# Autodesk Inventor assembly: Sessao7_02_04_2025_999_0001
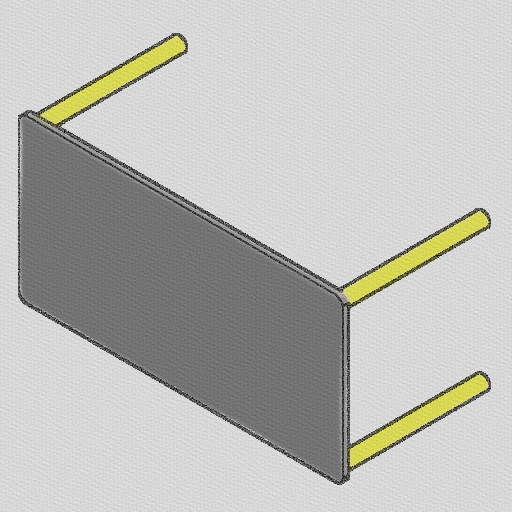
[picture p0: Inventor's stored thumbnail of the model, 512x512]
Saved by Autodesk Inventor 2025.2 (Build 292293000, 293)
## iProperties
Created: 2025-04-02
Part Number: Sessao7_02_04_2025_999_0001
Document SubType Name: Assembly
Designer: lucas
Author: lucas
## Documents named in this file (3)
- C:\Users\lucas\OneDrive\Documentos\Documentos\Gustavo\Mozangao\Robotica_Fundamentos\Inventor\Sessao7_02_04_2025\Sessao7_02_04_2025_999_0001.iam
- C:\Users\lucas\OneDrive\Documentos\Documentos\Gustavo\Mozangao\Robotica_Fundamentos\Inventor\Sessao7_02_04_2025\Sessao7_02_04_2025_0001_001.ipt
- C:\Users\lucas\OneDrive\Documentos\Documentos\Gustavo\Mozangao\Robotica_Fundamentos\Inventor\Sessao7_02_04_2025\Sessao7_02_04_2025_0002_001.ipt
## Components (5 placed, 2 different names)
1. Sessao7_02_04_2025_0001_001:1 — Alinhado:1, Alinhado:2, Alinhado:3, Coincidente:1, Coincidente:2, Coincidente:3, Coincidente:4, Coincidente:5, Alinhado:10, Coincidente:6, Coincidente:7, Coincidente:8, Coincidente:9
2. Sessao7_02_04_2025_0002_001:1 — Coincidente:1, Alinhado:6, Alinhado:7, Alinhado:8, Simetria:1, Simetria:3, Coincidente:5, Alinhado:10, Coincidente:9
3. Sessao7_02_04_2025_0002_001:2 — Coincidente:3, Alinhado:9, Simetria:2, Coincidente:7
4. Sessao7_02_04_2025_0002_001:3 — Coincidente:4, Alinhado:6, Alinhado:7, Simetria:1, Alinhado:9, Simetria:2, Coincidente:8
5. Sessao7_02_04_2025_0002_001:4 — Coincidente:2, Alinhado:8, Simetria:3, Coincidente:6
## Relationships (20: Mate 9, Flush 8, Symmetry 3)
- Alinhado:1 [Flush]: Sessao7_02_04_2025_0001_001:1
- Alinhado:2 [Flush]: Sessao7_02_04_2025_0001_001:1
- Alinhado:3 [Flush]: Sessao7_02_04_2025_0001_001:1
- Coincidente:1 [Mate]: Sessao7_02_04_2025_0001_001:1 ↔ Sessao7_02_04_2025_0002_001:1
- Coincidente:2 [Mate]: Sessao7_02_04_2025_0001_001:1 ↔ Sessao7_02_04_2025_0002_001:4
- Coincidente:3 [Mate]: Sessao7_02_04_2025_0001_001:1 ↔ Sessao7_02_04_2025_0002_001:2
- Coincidente:4 [Mate]: Sessao7_02_04_2025_0001_001:1 ↔ Sessao7_02_04_2025_0002_001:3
- Alinhado:6 [Flush]: Sessao7_02_04_2025_0002_001:1 ↔ Sessao7_02_04_2025_0002_001:3
- Alinhado:7 [Flush]: Sessao7_02_04_2025_0002_001:1 ↔ Sessao7_02_04_2025_0002_001:3
- Alinhado:8 [Flush]: Sessao7_02_04_2025_0002_001:1 ↔ Sessao7_02_04_2025_0002_001:4
- Simetria:1 [Symmetry]: Sessao7_02_04_2025_0002_001:1 ↔ Sessao7_02_04_2025_0002_001:3
- Alinhado:9 [Flush]: Sessao7_02_04_2025_0002_001:2 ↔ Sessao7_02_04_2025_0002_001:3
- Simetria:2 [Symmetry]: Sessao7_02_04_2025_0002_001:2 ↔ Sessao7_02_04_2025_0002_001:3
- Simetria:3 [Symmetry]: Sessao7_02_04_2025_0002_001:1 ↔ Sessao7_02_04_2025_0002_001:4
- Coincidente:5 [Mate] (-50 mm): Sessao7_02_04_2025_0001_001:1 ↔ Sessao7_02_04_2025_0002_001:1
- Alinhado:10 [Flush] (50 mm): Sessao7_02_04_2025_0001_001:1 ↔ Sessao7_02_04_2025_0002_001:1
- Coincidente:6 [Mate]: Sessao7_02_04_2025_0001_001:1 ↔ Sessao7_02_04_2025_0002_001:4
- Coincidente:7 [Mate]: Sessao7_02_04_2025_0001_001:1 ↔ Sessao7_02_04_2025_0002_001:2
- Coincidente:8 [Mate]: Sessao7_02_04_2025_0001_001:1 ↔ Sessao7_02_04_2025_0002_001:3
- Coincidente:9 [Mate]: Sessao7_02_04_2025_0001_001:1 ↔ Sessao7_02_04_2025_0002_001:1
